# Autodesk Inventor assembly: montagem-arcade
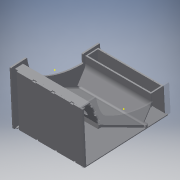
[picture p0: Inventor's stored thumbnail of the model, 180x180]
Saved by Autodesk Inventor 2016 (Build 200138000, 138)
## iProperties
Created: 2017-06-05
Part Number: montagem-arcade
Material: Genérico
Document SubType Name: Assembly
Designer: Fabio
Author: Fabio
## Documents named in this file (15)
- C:\dev\arcade\montagem-arcade.iam
- C:\dev\arcade\lateral.ipt
- C:\dev\arcade\traseira.ipt
- C:\dev\arcade\BASE.ipt
- C:\dev\arcade\frente inferior.ipt
- C:\dev\arcade\controles.ipt
- C:\dev\arcade\junta controler.ipt
- C:\dev\arcade\fechamento superior.ipt
- C:\dev\arcade\letreiro.ipt
- C:\dev\arcade\fechamento inferior.ipt
- C:\dev\arcade\junta auto falante.ipt
- C:\dev\arcade\placa auto falante.ipt
- C:\dev\arcade\tela.ipt
- C:\dev\arcade\juncao controle tela.ipt
- C:\dev\arcade\juncao tela - som.ipt
## Components (15 placed, 14 different names)
1. lateral:1 — Mate:4, Mate:6
2. lateral:2 — Mate:3, Flush:5, Flush:6, Mate:9, Mate:12, Mate:15
3. traseira:1 — Mate:3, Flush:5, Flush:6, Mate:4, Mate:5, Flush:7, Mate:7, Mate:14, Flush:10
4. BASE:1 — Mate:5, Flush:7, Mate:6, Mate:7, Mate:8, Flush:8
5. frente inferior:1 — Mate:8, Flush:8, Mate:9, Mate:10, Mate:11
6. junta controler:1 — Mate:10, Mate:11, Mate:12, Mate:13, Flush:9
7. controles:1 — Mate:13, Flush:9, Alinhamento:19
8. fechamento superior:1 — Mate:14, Flush:10, Mate:15, Flush:11, Flush:12, Mate:16
9. letreiro:1 — Flush:11, Flush:12, Mate:16, Flush:13, Mate:17, Flush:14
10. fechamento inferior:1 — Flush:13, Mate:17, Flush:14, Alinhamento:16, Coincidência:19, Alinhamento:17
11. junta auto falante:1 — Coincidência:19, Alinhamento:17, Coincidência:20, Alinhamento:18
12. placa auto falante:1 — Alinhamento:16, Coincidência:20, Alinhamento:18
13. tela:1 — Alinhamento:20
14. juncao controle tela:1 — Alinhamento:19, Alinhamento:20
15. juncao tela - som:1
## Relationships (32: Mate 17, Flush 15)
- Mate:3: lateral:2 ↔ traseira:1
- Flush:5: lateral:2 ↔ traseira:1
- Flush:6 (10 mm): lateral:2 ↔ traseira:1
- Mate:4: lateral:1 ↔ traseira:1
- Mate:5 (-4 mm): traseira:1 ↔ BASE:1
- Flush:7: traseira:1 ↔ BASE:1
- Mate:6: lateral:1 ↔ BASE:1
- Mate:7 (-4 mm): traseira:1 ↔ BASE:1
- Mate:8 (-8 mm): BASE:1 ↔ frente inferior:1
- Flush:8: BASE:1 ↔ frente inferior:1
- Mate:9 (-8 mm): lateral:2 ↔ frente inferior:1
- Mate:10: frente inferior:1 ↔ junta controler:1
- Mate:11: frente inferior:1 ↔ junta controler:1
- Mate:12: lateral:2 ↔ junta controler:1
- Mate:13: junta controler:1 ↔ controles:1
- Flush:9 (-8 mm): junta controler:1 ↔ controles:1
- Mate:14 (-4 mm): traseira:1 ↔ fechamento superior:1
- Flush:10: traseira:1 ↔ fechamento superior:1
- Mate:15: lateral:2 ↔ fechamento superior:1
- Flush:11: fechamento superior:1 ↔ letreiro:1
- Flush:12: fechamento superior:1 ↔ letreiro:1
- Mate:16 (-4 mm): fechamento superior:1 ↔ letreiro:1
- Flush:13: letreiro:1 ↔ fechamento inferior:1
- Mate:17 (-4 mm): letreiro:1 ↔ fechamento inferior:1
- Flush:14: letreiro:1 ↔ fechamento inferior:1
- Alinhamento:16 [Flush]: fechamento inferior:1 ↔ placa auto falante:1
- Coincidência:19 [Mate]: fechamento inferior:1 ↔ junta auto falante:1
- Alinhamento:17 [Flush]: fechamento inferior:1 ↔ junta auto falante:1
- Coincidência:20 [Mate]: junta auto falante:1 ↔ placa auto falante:1
- Alinhamento:18 [Flush]: junta auto falante:1 ↔ placa auto falante:1
- Alinhamento:19 [Flush]: controles:1 ↔ juncao controle tela:1
- Alinhamento:20 [Flush]: tela:1 ↔ juncao controle tela:1
